# Autodesk Inventor assembly: Shield_top_sestava
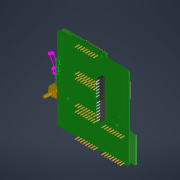
[picture p0: Inventor's stored thumbnail of the model, 180x180]
Saved by Autodesk Inventor 2022 (Build 260153000, 153)
## iProperties
Created: 2022-03-30
Part Number: Shield_top_sestava
Document SubType Name: Assembly
Designer: dvorakj
Author: dvorakj
## Documents named in this file (8)
- C:\Users\dvorakj\Documents\Inventor\Bakalarka\altium export\Shield_top\Shield_top_sestava.iam
- C:\Users\dvorakj\Documents\Inventor\Bakalarka\altium export\Shield_top\Shield_top_pcb.ipt
- C:\Users\dvorakj\Documents\Inventor\Bakalarka\Clicks\DHT22\DHT_sestava.iam
- C:\Users\dvorakj\Documents\Inventor\Bakalarka\Clicks\GNSS\GNSS_sestava.iam
- C:\Users\dvorakj\Documents\Inventor\Bakalarka\Clicks\tRF\tRF sestava.iam
- C:\Users\dvorakj\Documents\Inventor\Bakalarka\Clicks\MPU\MPU.iam
- C:\Users\dvorakj\Documents\Inventor\Bakalarka\MS5607\MS5607.iam
- C:\Users\dvorakj\Documents\Inventor\Bakalarka\Openlog\openlog sestava.iam
## Components (7 placed, 7 different names)
1. Shield_top_pcb:1 — Insert:1, Mate:1, Mate:2, Mate:3, Mate:4, Angle:1, Angle:2, Angle:3, Angle:5, Angle:6
2. DHT_sestava:1 [sub-assembly] — Flush:5, Flush:6, Flush:7, Mate:2, Angle:3
3. GNSS_sestava:1 [sub-assembly] — Flush:6, Flush:7, Flush:8, Mate:1, Angle:6
4. tRF sestava:1 [sub-assembly] — Flush:4, Flush:5, Flush:8, Flush:9, Insert:1, Angle:5
5. MPU:1 [sub-assembly] — Flush:1, Flush:2, Flush:3, Flush:4, Flush:9, Flush:10
6. MS5607:1 [sub-assembly] — Flush:3, Flush:10, Flush:11, Mate:4, Angle:1
7. openlog sestava:1 [sub-assembly] — Flush:1, Flush:2, Flush:11, Mate:3, Angle:2
## Relationships (21: Flush 11, Angle 5, Mate 4, Insert 1)
- Flush:1: MPU:1 ↔ openlog sestava:1
- Flush:2: MPU:1 ↔ openlog sestava:1
- Flush:3: MPU:1 ↔ MS5607:1
- Flush:4: tRF sestava:1 ↔ MPU:1
- Flush:5: DHT_sestava:1 ↔ tRF sestava:1
- Flush:6: DHT_sestava:1 ↔ GNSS_sestava:1
- Flush:7: DHT_sestava:1 ↔ GNSS_sestava:1
- Flush:8: GNSS_sestava:1 ↔ tRF sestava:1
- Flush:9: tRF sestava:1 ↔ MPU:1
- Flush:10: MPU:1 ↔ MS5607:1
- Flush:11: MS5607:1 ↔ openlog sestava:1
- Insert:1: Shield_top_pcb:1 ↔ tRF sestava:1
- Mate:1: Shield_top_pcb:1 ↔ GNSS_sestava:1
- Mate:2: Shield_top_pcb:1 ↔ DHT_sestava:1
- Mate:3: Shield_top_pcb:1 ↔ openlog sestava:1
- Mate:4: Shield_top_pcb:1 ↔ MS5607:1
- Angle:1 (0 deg): Shield_top_pcb:1 ↔ MS5607:1
- Angle:2 (0 deg): Shield_top_pcb:1 ↔ openlog sestava:1
- Angle:3 (0 deg): Shield_top_pcb:1 ↔ DHT_sestava:1
- Angle:5 (0 deg): Shield_top_pcb:1 ↔ tRF sestava:1
- Angle:6 (-90 deg): Shield_top_pcb:1 ↔ GNSS_sestava:1
